# Autodesk Inventor assembly: IO Board
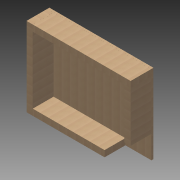
[picture p0: Inventor's stored thumbnail of the model, 180x180]
Saved by Autodesk Inventor 2015 (Build 190159000, 159)
## iProperties
Created: 2015-01-25
Part Number: IO Board
Document SubType Name: Assembly
Designer: Michael7
Author: Michael7
## Documents named in this file (6)
- C:\Users\Michael7\Documents\IO MK 1\IO Board.iam
- C:\Users\Michael7\Documents\IO MK 1\Base.ipt
- C:\Users\Michael7\Documents\IO MK 1\6 in side.ipt
- C:\Users\Michael7\Documents\IO MK 1\8.625 in side.ipt
- C:\Users\Michael7\Documents\IO MK 1\9.5 in side.ipt
- C:\Users\Michael7\Documents\IO MK 1\11.75 in side.ipt
## Components (5 placed, 5 different names)
1. Base:1 — Mate:1, Mate:2, Mate:3, Mate:4, Mate:5, Mate:7, Mate:8, Mate:9, Mate:10, Mate:11
2. 6 in side:1 — Mate:1, Mate:2, Mate:6
3. 8.625 in side:1 — Mate:10, Mate:11, Mate:12
4. 9.5 in side:1 — Mate:7, Mate:8, Mate:9, Mate:12
5. 11.75 in side:1 — Mate:3, Mate:4, Mate:5, Mate:6
## Relationships (12: Mate 12)
- Mate:1: Base:1 ↔ 6 in side:1
- Mate:2: Base:1 ↔ 6 in side:1
- Mate:3: Base:1 ↔ 11.75 in side:1
- Mate:4: Base:1 ↔ 11.75 in side:1
- Mate:5: Base:1 ↔ 11.75 in side:1
- Mate:6: 6 in side:1 ↔ 11.75 in side:1
- Mate:7: Base:1 ↔ 9.5 in side:1
- Mate:8: Base:1 ↔ 9.5 in side:1
- Mate:9: Base:1 ↔ 9.5 in side:1
- Mate:10: Base:1 ↔ 8.625 in side:1
- Mate:11: Base:1 ↔ 8.625 in side:1
- Mate:12: 8.625 in side:1 ↔ 9.5 in side:1
